# Autodesk Inventor assembly: Carriage Assembly
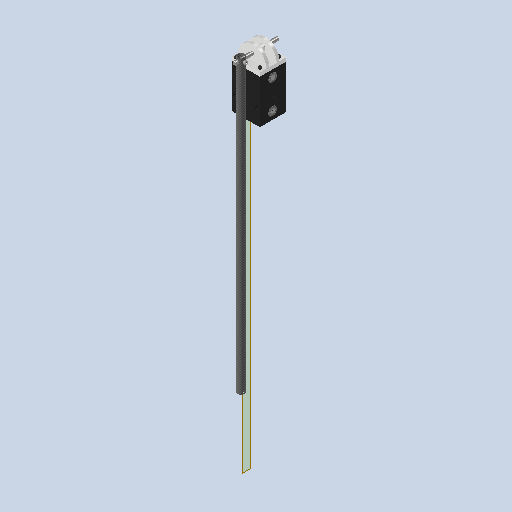
[picture p0: Inventor's stored thumbnail of the model, 512x512]
Saved by Autodesk Inventor 2023 (Build 270158000, 158)
## iProperties
Created: 2023-02-06
Part Number: Carriage Assembly
Document SubType Name: Assembly
Designer: mbear
Author: mbear
## Documents named in this file (12)
- C:\Users\mbear\OneDrive\Documents\Inventor\Inverted Pendulum\Carriage Assembly.iam
- C:\Users\mbear\OneDrive\Documents\Inventor\Inverted Pendulum\Dry Bearing.ipt
- C:\Users\mbear\OneDrive\Documents\Inventor\Inverted Pendulum\Carriage Design Left.ipt
- C:\Users\mbear\OneDrive\Documents\Inventor\Inverted Pendulum\Carriage Top.ipt
- C:\Users\mbear\OneDrive\Documents\Inventor\Inverted Pendulum\Carriage Axle V1.ipt
- C:\Users\mbear\OneDrive\Documents\Inventor\Inverted Pendulum\Pendulum Tubing.ipt
- C:\Users\mbear\OneDrive\Documents\Inventor\Inverted Pendulum\Carriage Axle Set Screw Holder.ipt
- C:\Users\mbear\OneDrive\Documents\Inventor\Inverted Pendulum\Hex_Socket_M3x16.ipt
- C:\Users\mbear\OneDrive\Documents\Inventor\Inverted Pendulum\M3 Nyloc Nut.ipt
- C:\Users\mbear\OneDrive\Documents\Inventor\Inverted Pendulum\M3 Square Nut.ipt
- C:\Users\mbear\OneDrive\Documents\Inventor\Inverted Pendulum\Carriage Design Right.ipt
- C:\Users\mbear\OneDrive\Documents\Inventor\Inverted Pendulum\Hex_Socket_M3x14.ipt
## Components (24 placed, 11 different names)
1. Dry Bearing:1
2. Dry Bearing:2
3. Dry Bearing:3
4. Dry Bearing:4
5. Carriage Design Left:1 — Mate:2, Insert:11, Angle:2, Insert:12, Angle:3, Mate:9, Flush:6, Flush:7, Insert:13, Insert:14, Angle:5
6. Carriage Top:1 — Mate:2, Insert:5, Mate:3, Insert:6, Insert:7, Insert:8, Insert:9, Angle:1, Mate:10, Flush:8, Flush:9
7. Carriage Axle V1:1 — Mate:3, Mate:4, Mate:5, Mate:6
8. Pendulum Tubing:1 — Mate:5, Mate:6, Mate:7, Angle:1, Flush:5
9. Carriage Axle Set Screw Holder:1 — Insert:5, Mate:4
10. Hex_Socket_M3x16:1 — Insert:9
11. Hex_Socket_M3x16:2 — Insert:8
12. Hex_Socket_M3x16:3 — Insert:6
13. Hex_Socket_M3x16:4 — Insert:7
14. Hex_Socket_M3x16:5 — Mate:7, Mate:8, Insert:10
15. M3 Nyloc Nut:1 — Insert:10
16. M3 Square Nut:1
17. M3 Square Nut:2
18. M3 Square Nut:3 — Insert:12, Angle:3
19. M3 Square Nut:4 — Insert:11, Angle:2
20. Carriage Design Right:1 — Mate:9, Flush:6, Flush:7, Insert:15, Angle:4, Insert:16, Mate:10, Flush:8, Flush:9
21. Hex_Socket_M3x14:1 — Insert:13
22. Hex_Socket_M3x14:2 — Insert:14
23. M3 Square Nut:5 — Insert:15, Angle:4
24. M3 Square Nut:6 — Insert:16, Angle:5
## Relationships (31: Insert 12, Mate 9, Angle 5, Flush 5)
- Mate:2: Carriage Design Left:1 ↔ Carriage Top:1
- Insert:5: Carriage Top:1 ↔ Carriage Axle Set Screw Holder:1
- Mate:3: Carriage Top:1 ↔ Carriage Axle V1:1
- Mate:4: Carriage Axle V1:1 ↔ Carriage Axle Set Screw Holder:1
- Mate:5: Carriage Axle V1:1 ↔ Pendulum Tubing:1
- Mate:6: Carriage Axle V1:1 ↔ Pendulum Tubing:1
- Insert:6: Carriage Top:1 ↔ Hex_Socket_M3x16:3
- Insert:7: Carriage Top:1 ↔ Hex_Socket_M3x16:4
- Insert:8: Carriage Top:1 ↔ Hex_Socket_M3x16:2
- Insert:9: Carriage Top:1 ↔ Hex_Socket_M3x16:1
- Mate:7: Pendulum Tubing:1 ↔ Hex_Socket_M3x16:5
- Angle:1 (0 deg): Carriage Top:1 ↔ Pendulum Tubing:1
- Flush:5 (6.35 mm): Pendulum Tubing:1
- Mate:8: Hex_Socket_M3x16:5
- Insert:10 (0.508 mm): Hex_Socket_M3x16:5 ↔ M3 Nyloc Nut:1
- Insert:11: Carriage Design Left:1 ↔ M3 Square Nut:4
- Angle:2 (0 deg): Carriage Design Left:1 ↔ M3 Square Nut:4
- Insert:12: Carriage Design Left:1 ↔ M3 Square Nut:3
- Angle:3 (0 deg): Carriage Design Left:1 ↔ M3 Square Nut:3
- Mate:9: Carriage Design Left:1 ↔ Carriage Design Right:1
- Flush:6: Carriage Design Left:1 ↔ Carriage Design Right:1
- Flush:7: Carriage Design Left:1 ↔ Carriage Design Right:1
- Insert:13: Carriage Design Left:1 ↔ Hex_Socket_M3x14:1
- Insert:14: Carriage Design Left:1 ↔ Hex_Socket_M3x14:2
- Insert:15: Carriage Design Right:1 ↔ M3 Square Nut:5
- Angle:4 (0 deg): Carriage Design Right:1 ↔ M3 Square Nut:5
- Insert:16: Carriage Design Right:1 ↔ M3 Square Nut:6
- Angle:5 (0 deg): Carriage Design Left:1 ↔ M3 Square Nut:6
- Mate:10: Carriage Top:1 ↔ Carriage Design Right:1
- Flush:8: Carriage Top:1 ↔ Carriage Design Right:1
- Flush:9: Carriage Top:1 ↔ Carriage Design Right:1
